# Autodesk Inventor assembly: Electrical Ring
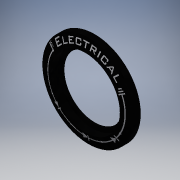
[picture p0: Inventor's stored thumbnail of the model, 180x180]
Saved by Autodesk Inventor 2016 (Build 200138000, 138)
## iProperties
Created: 2015-06-02
Part Number: Electrical Ring
Document SubType Name: Assembly
Designer: Spooner
Author: Spooner
## Documents named in this file (4)
- C:\Users\Spooner\Documents\Inventor\2016 RoboCat\Electrical Ring.iam
- C:\Users\Spooner\Documents\Inventor\2016 RoboCat\Team Pin Electrical.ipt
- C:\Users\Spooner\Documents\Inventor\2016 RoboCat\Team Pin Electrical-circuit.ipt
- C:\Users\Spooner\Documents\Inventor\2016 RoboCat\Team Pin Electrical-Text.ipt
## Components (3 placed, 3 different names)
1. Team Pin Electrical:1 — Mate:10, Mate:11, Mate:12, Mate:13, Mate:14, Mate:15
2. Team Pin Electrical-circuit:1 — Mate:10, Mate:14, Mate:15
3. Team Pin Electrical-Text:1 — Mate:11, Mate:12, Mate:13
## Relationships (6: Mate 6)
- Mate:10: Team Pin Electrical:1 ↔ Team Pin Electrical-circuit:1
- Mate:11: Team Pin Electrical:1 ↔ Team Pin Electrical-Text:1
- Mate:12: Team Pin Electrical:1 ↔ Team Pin Electrical-Text:1
- Mate:13: Team Pin Electrical:1 ↔ Team Pin Electrical-Text:1
- Mate:14: Team Pin Electrical:1 ↔ Team Pin Electrical-circuit:1
- Mate:15: Team Pin Electrical:1 ↔ Team Pin Electrical-circuit:1
